# Autodesk Inventor assembly: module_icicles26
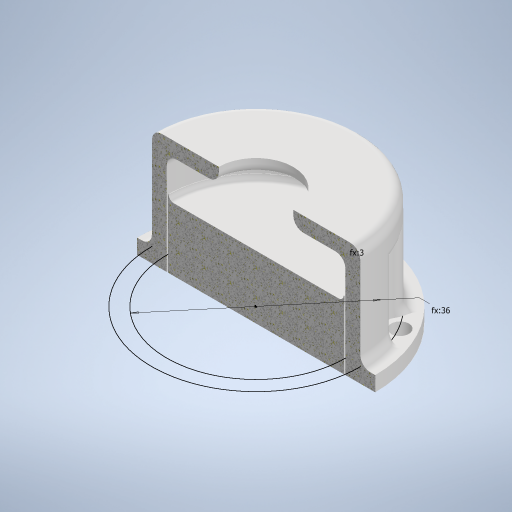
[picture p0: Inventor's stored thumbnail of the model, 512x512]
Saved by Autodesk Inventor 2023 (Build 270158000, 158)
## iProperties
Created: 2022-10-31
Part Number: module_icicles26
Document SubType Name: Assembly
Designer: incep
Author: incep
## Documents named in this file (3)
- C:\Users\incep\OneDrive\Desktop\Laser Cutter Things\ModularUhOhChair\module_icicles26.iam
- C:\Users\incep\OneDrive\Desktop\Laser Cutter Things\ModularUhOhChair\Module_top_Icicles26.ipt
- C:\Users\incep\OneDrive\Desktop\Laser Cutter Things\ModularUhOhChair\Module_bottom_Icicles26_v2.ipt
## Components (2 placed, 2 different names)
1. Module_top_Icicles26:1 — Mate:1, Flush:1, Mate:2, Mate:3
2. Module_bottom_Icicles26_v2:1 — Mate:1, Flush:1
## Relationships (4: Mate 3, Flush 1)
- Mate:1: Module_top_Icicles26:1 ↔ Module_bottom_Icicles26_v2:1
- Flush:1: Module_top_Icicles26:1 ↔ Module_bottom_Icicles26_v2:1
- Mate:2: Module_top_Icicles26:1
- Mate:3: Module_top_Icicles26:1
